# Autodesk Inventor assembly: boxanddrawer
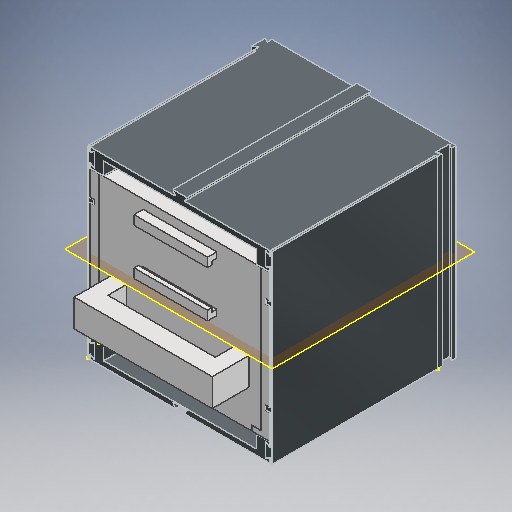
[picture p0: Inventor's stored thumbnail of the model, 512x512]
Saved by Autodesk Inventor 2025.2 (Build 292293000, 293)
## iProperties
Created: 2025-03-25
Part Number: boxanddrawer
Document SubType Name: Assembly
Designer: Alex
Author: Alex
## Documents named in this file (3)
- C:\Shared\alex-bartella-schoolwork\4b03\dr3\v2\boxanddrawer.iam
- C:\Shared\alex-bartella-schoolwork\4b03\dr3\v2\boxassem.iam
- C:\Shared\alex-bartella-schoolwork\4b03\dr3\v2\drawerassem.iam
## Components (2 placed, 2 different names)
1. boxassem:1 [sub-assembly] — Mate:1, Mate:5, Mate:6, Mate:7, Mate:8, Mate:9
2. drawerassem:1 [sub-assembly] — Mate:7, Mate:8, Mate:9
## Relationships (6: Mate 6)
- Mate:1: boxassem:1
- Mate:5: boxassem:1
- Mate:6: boxassem:1
- Mate:7 (0.2 mm): boxassem:1 ↔ drawerassem:1
- Mate:8 (0.2 mm): boxassem:1 ↔ drawerassem:1
- Mate:9: boxassem:1 ↔ drawerassem:1
## Named parameters: tol = 0.1 mm
